# Autodesk Inventor assembly: centre wing
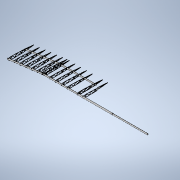
[picture p0: Inventor's stored thumbnail of the model, 180x180]
Saved by Autodesk Inventor 2022 (Build 260153000, 153)
## iProperties
Created: 2021-03-09
Part Number: centre wing
Document SubType Name: Assembly
Designer: Ferdinand Hubbard
Author: Ferdinand Hubbard
## Documents named in this file (8)
- C:\Users\Ferdinand Hubbard\Desktop\solar-plane\cad\right wing section.iam
- C:\Users\Ferdinand Hubbard\Desktop\solar-plane\cad\15mm tube.ipt
- C:\Users\Ferdinand Hubbard\Desktop\solar-plane\cad\angle connector 16 mm.ipt
- C:\Users\Ferdinand Hubbard\Desktop\solar-plane\cad\18mm tube.ipt
- C:\Users\Ferdinand Hubbard\Desktop\solar-plane\cad\airfoils\full airfoil\full airfoil blueprint 16 mm.ipt
- C:\Users\Ferdinand Hubbard\Desktop\solar-plane\cad\airfoils\full airfoil adjacent to aileron\full adjacent to aileron airfoil 16 mm.ipt
- C:\Users\Ferdinand Hubbard\Desktop\solar-plane\cad\airfoils\front half aileron\front half airfoil 19 mm.ipt
- C:\Users\Ferdinand Hubbard\Desktop\solar-plane\cad\airfoils\back half aileron\back half aileron airfoil 19mm.ipt
## Components (23 placed, 7 different names)
1. angle connector 16 mm:1 — Mate:1, Mate:2, Mate:3, Mate:4, Angle:3
2. angle connector 16 mm:2 — Angle:5
3. 15mm tube:1 — Mate:1, Mate:2, Flush:1, Mate:32, Angle:2, Flush:4, Flush:10
4. 15mm tube:5 — Flush:5, Angle:6, Mate:50, Flush:12
5. 15mm tube:2 — Mate:3, Mate:4, Mate:5, Mate:6, Flush:3, Mate:49, Angle:4
6. 15mm tube:3 — Mate:7, Mate:8
7. 18mm tube:1 — Mate:5, Mate:6, Mate:7, Mate:8
8. full airfoil blueprint 16 mm:1 — Mate:9, Mate:10, Mate:11, Flush:1, Mate:32, Mate:33, Flush:2, Angle:1, Angle:2
9. full airfoil blueprint 16 mm:2 — Mate:9, Mate:10, Mate:11, Mate:15, Mate:16, Mate:17
10. full airfoil blueprint 16 mm:3 — Mate:15, Mate:16, Mate:17
11. full airfoil blueprint 16 mm:4 — Mate:21, Mate:22, Mate:23
12. full airfoil blueprint 16 mm:5 — Mate:21, Mate:22, Mate:23
13. full airfoil blueprint 16 mm:6 — Mate:91, Mate:92
14. 15mm tube:4 — Mate:33, Flush:2, Angle:1, Flush:4, Flush:9
15. full airfoil blueprint 16 mm:7 — Flush:3, Mate:49, Flush:5, Angle:3, Angle:4, Angle:5, Angle:6, Mate:50
16. full airfoil blueprint 16 mm:8
17. full airfoil blueprint 16 mm:9
18. full airfoil blueprint 16 mm:10
19. full airfoil blueprint 16 mm:11 — Mate:93, Flush:11
20. full airfoil blueprint 16 mm:20 — Mate:91, Mate:92, Flush:9, Flush:10
21. full adjacent to aileron airfoil 16 mm:1 — Mate:93, Flush:11, Flush:12, Mate:94, Mate:95, Mate:96, Flush:13
22. front half airfoil 19 mm:1 — Mate:94, Mate:95
23. back half aileron airfoil 19mm:1 — Mate:96, Flush:13
## Relationships (63: Mate 47, Flush 10, Angle 6)
- Mate:1: angle connector 16 mm:1 ↔ 15mm tube:1
- Mate:2: angle connector 16 mm:1 ↔ 15mm tube:1
- Mate:3: angle connector 16 mm:1 ↔ 15mm tube:2
- Mate:4: angle connector 16 mm:1 ↔ 15mm tube:2
- Mate:5: 15mm tube:2 ↔ 18mm tube:1
- Mate:6: 15mm tube:2 ↔ 18mm tube:1
- Mate:7: 15mm tube:3 ↔ 18mm tube:1
- Mate:8: 15mm tube:3 ↔ 18mm tube:1
- Mate:9 (80 mm): full airfoil blueprint 16 mm:1 ↔ full airfoil blueprint 16 mm:2
- Mate:10: full airfoil blueprint 16 mm:1 ↔ full airfoil blueprint 16 mm:2
- Mate:11: full airfoil blueprint 16 mm:1 ↔ full airfoil blueprint 16 mm:2
- [Mate] (80 mm): full airfoil blueprint 16 mm:3 ↔ full airfoil blueprint 16 mm:4
- [Mate]: full airfoil blueprint 16 mm:3 ↔ full airfoil blueprint 16 mm:4
- [Mate]: full airfoil blueprint 16 mm:3 ↔ full airfoil blueprint 16 mm:4
- Mate:15: full airfoil blueprint 16 mm:2 ↔ full airfoil blueprint 16 mm:3
- Mate:16: full airfoil blueprint 16 mm:2 ↔ full airfoil blueprint 16 mm:3
- Mate:17 (80 mm): full airfoil blueprint 16 mm:2 ↔ full airfoil blueprint 16 mm:3
- Flush:1 (12 mm): 15mm tube:1 ↔ full airfoil blueprint 16 mm:1
- [Mate] (80 mm): full airfoil blueprint 16 mm:5 ↔ full airfoil blueprint 16 mm:6
- [Mate]: full airfoil blueprint 16 mm:5 ↔ full airfoil blueprint 16 mm:6
- [Mate]: full airfoil blueprint 16 mm:5 ↔ full airfoil blueprint 16 mm:6
- Mate:21 (80 mm): full airfoil blueprint 16 mm:4 ↔ full airfoil blueprint 16 mm:5
- Mate:22: full airfoil blueprint 16 mm:4 ↔ full airfoil blueprint 16 mm:5
- Mate:23: full airfoil blueprint 16 mm:4 ↔ full airfoil blueprint 16 mm:5
- [Mate]: angle connector 16 mm:2 ↔ 15mm tube:4
- [Mate]: angle connector 16 mm:2 ↔ 15mm tube:4
- Mate:32: 15mm tube:1 ↔ full airfoil blueprint 16 mm:1
- Mate:33: full airfoil blueprint 16 mm:1 ↔ 15mm tube:4
- Flush:2 (12 mm): full airfoil blueprint 16 mm:1 ↔ 15mm tube:4
- [Mate] (80 mm): full airfoil blueprint 16 mm:7 ↔ full airfoil blueprint 16 mm:8
- [Mate]: full airfoil blueprint 16 mm:7 ↔ full airfoil blueprint 16 mm:8
- [Mate]: full airfoil blueprint 16 mm:7 ↔ full airfoil blueprint 16 mm:8
- [Mate] (80 mm): full airfoil blueprint 16 mm:9 ↔ full airfoil blueprint 16 mm:10
- [Mate]: full airfoil blueprint 16 mm:9 ↔ full airfoil blueprint 16 mm:10
- [Mate]: full airfoil blueprint 16 mm:9 ↔ full airfoil blueprint 16 mm:10
- [Mate]: full airfoil blueprint 16 mm:8 ↔ full airfoil blueprint 16 mm:9
- [Mate]: full airfoil blueprint 16 mm:8 ↔ full airfoil blueprint 16 mm:9
- [Mate] (80 mm): full airfoil blueprint 16 mm:8 ↔ full airfoil blueprint 16 mm:9
- [Mate] (80 mm): full airfoil blueprint 16 mm:10 ↔ full airfoil blueprint 16 mm:11
- [Mate]: full airfoil blueprint 16 mm:10 ↔ full airfoil blueprint 16 mm:11
- [Mate]: full airfoil blueprint 16 mm:10 ↔ full airfoil blueprint 16 mm:11
- Angle:1 (270 deg): full airfoil blueprint 16 mm:1 ↔ 15mm tube:4
- Angle:2 (270 deg): 15mm tube:1 ↔ full airfoil blueprint 16 mm:1
- Flush:3 (12 mm): 15mm tube:2 ↔ full airfoil blueprint 16 mm:7
- Mate:49: 15mm tube:2 ↔ full airfoil blueprint 16 mm:7
- Flush:4: 15mm tube:1 ↔ 15mm tube:4
- Flush:5 (12 mm): 15mm tube:5 ↔ full airfoil blueprint 16 mm:7
- Angle:3 (0 deg): angle connector 16 mm:1 ↔ full airfoil blueprint 16 mm:7
- Angle:4 (180 deg): 15mm tube:2 ↔ full airfoil blueprint 16 mm:7
- Angle:5 (0 deg): angle connector 16 mm:2 ↔ full airfoil blueprint 16 mm:7
- Angle:6 (0 deg): 15mm tube:5 ↔ full airfoil blueprint 16 mm:7
- Mate:50: 15mm tube:5 ↔ full airfoil blueprint 16 mm:7
- Mate:91: full airfoil blueprint 16 mm:6 ↔ full airfoil blueprint 16 mm:20
- Mate:92: full airfoil blueprint 16 mm:6 ↔ full airfoil blueprint 16 mm:20
- Flush:9 (12 mm): 15mm tube:4 ↔ full airfoil blueprint 16 mm:20
- Flush:10 (12 mm): 15mm tube:1 ↔ full airfoil blueprint 16 mm:20
- Mate:93: full airfoil blueprint 16 mm:11 ↔ full adjacent to aileron airfoil 16 mm:1
- Flush:11: full airfoil blueprint 16 mm:11 ↔ full adjacent to aileron airfoil 16 mm:1
- Flush:12 (12 mm): 15mm tube:5 ↔ full adjacent to aileron airfoil 16 mm:1
- Mate:94: full adjacent to aileron airfoil 16 mm:1 ↔ front half airfoil 19 mm:1
- Mate:95: full adjacent to aileron airfoil 16 mm:1 ↔ front half airfoil 19 mm:1
- Mate:96: full adjacent to aileron airfoil 16 mm:1 ↔ back half aileron airfoil 19mm:1
- Flush:13: full adjacent to aileron airfoil 16 mm:1 ↔ back half aileron airfoil 19mm:1
## Named parameters: d220_d217 = 80 mm, d221_d218 = 0 mm, d222_d219 = 0 mm, d227_d220_d217 = 80 mm, d228_d221_d218 = 0 mm, d229_d222_d219 = 0 mm, d233_d209 = 0 mm, d234_d210 = 0 mm, d244_d217 = 80 mm, d245_d218 = 0 mm, d246_d219 = 0 mm, d247_d220_d217 = 80 mm, d248_d221_d218 = 0 mm, d249_d222_d219 = 0 mm, d250_d223 = 0 mm, d251_d224 = 0 mm, d252_d225 = 80 mm, d256_d230 = 80 mm, d257_d231 = 0 mm, d258_d232 = 0 mm
